# Autodesk Inventor assembly: AM14U2+Long+FIXED
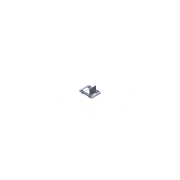
[picture p0: Inventor's stored thumbnail of the model, 180x180]
Saved by Autodesk Inventor 2015 (Build 190159000, 159)
## iProperties
Created: 2015-03-06
Part Number: AM14U2+Long+FIXED
Document SubType Name: Assembly
Designer: Kyle
Author: Kyle
Title: AM14U2 Long FIXED.STEP
Description: STEP AP214
Creation Date: 2015-01-13
Sending System: SolidWorks 2014
Preprocessor: SwSTEP 2.0
## Documents named in this file (5)
- C:\Users\Kyle\Documents\Inventor\ReDesign\Imported Components\AM14U2+Long+FIXED\AM14U2+Long+FIXED.iam
- C:\Users\Kyle\Documents\Inventor\ReDesign\Imported Components\AM14U2+Long+FIXED\AM14U2 Half Long.iam
- C:\Users\Kyle\Documents\Inventor\ReDesign\Wheel.ipt
- C:\Users\Kyle\Documents\Inventor\ReDesign\Toughbox+Nano+All+Shafts+v2.iam
- C:\Users\Kyle\Documents\Inventor\ReDesign\ControlBoard.ipt
## Components (9 placed, 5 different names)
1. AM14U2 Half Long_1 [sub-assembly] — Rotational:1, Mate:1, Mate:2, Mate:3, Rotational:3, Mate:6, Angle:2, Mate:9
2. AM14U2 Half Long_2 [sub-assembly] — Rotational:2, Mate:1, Mate:2, Mate:3, Rotational:4, Mate:4, Angle:1, Mate:8, Mate:11
3. Wheel:1 — Rotational:1, Mate:7
4. Wheel:2 — Rotational:2, Mate:5
5. Wheel:3 — Rotational:3
6. Wheel:4 — Rotational:4
7. Toughbox+Nano+All+Shafts+v2:1 [sub-assembly] — Mate:6, Mate:7, Angle:2
8. Toughbox+Nano+All+Shafts+v2:2 [sub-assembly] — Mate:4, Mate:5, Angle:1, Mate:10
9. ControlBoard:1 — Mate:8, Mate:9, Mate:10, Mate:11
## Relationships (17: Mate 11, RevoluteJoint 4, Angle 2)
- Rotational:1 [RevoluteJoint] (38.1 mm): AM14U2 Half Long_1 ↔ Wheel:1
- Rotational:2 [RevoluteJoint] (55.88 mm): AM14U2 Half Long_2 ↔ Wheel:2
- Mate:1: AM14U2 Half Long_1 ↔ AM14U2 Half Long_2
- Mate:2: AM14U2 Half Long_1 ↔ AM14U2 Half Long_2
- Mate:3: AM14U2 Half Long_1 ↔ AM14U2 Half Long_2
- Rotational:3 [RevoluteJoint] (57.15 mm): AM14U2 Half Long_1 ↔ Wheel:3
- Rotational:4 [RevoluteJoint] (55.88 mm): AM14U2 Half Long_2 ↔ Wheel:4
- Mate:4: AM14U2 Half Long_2 ↔ Toughbox+Nano+All+Shafts+v2:2
- Mate:5: Wheel:2 ↔ Toughbox+Nano+All+Shafts+v2:2
- Angle:1 (0 deg): AM14U2 Half Long_2 ↔ Toughbox+Nano+All+Shafts+v2:2
- Mate:6: AM14U2 Half Long_1 ↔ Toughbox+Nano+All+Shafts+v2:1
- Mate:7: Wheel:1 ↔ Toughbox+Nano+All+Shafts+v2:1
- Angle:2 (180 deg): AM14U2 Half Long_1 ↔ Toughbox+Nano+All+Shafts+v2:1
- Mate:8: AM14U2 Half Long_2 ↔ ControlBoard:1
- Mate:9: AM14U2 Half Long_1 ↔ ControlBoard:1
- Mate:10: Toughbox+Nano+All+Shafts+v2:2 ↔ ControlBoard:1
- Mate:11: AM14U2 Half Long_2 ↔ ControlBoard:1
